# Autodesk Inventor assembly: main_assy
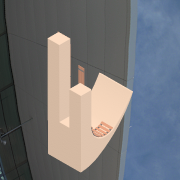
[picture p0: Inventor's stored thumbnail of the model, 180x180]
Saved by Autodesk Inventor 2019 (Build 230136000, 136)
## iProperties
Created: 2019-02-23
Part Number: main_assy
Document SubType Name: Assembly
Designer: gaincarlo
Author: gaincarlo
## Documents named in this file (9)
- D:\Giancarlo Bacchio\Documenti\00 - Progetti\30-Inventor\LaPanca-Baraca\main_assy.iam
- D:\Giancarlo Bacchio\Documenti\00 - Progetti\30-Inventor\LaPanca-Baraca\concrete_main.ipt
- D:\Giancarlo Bacchio\Documenti\00 - Progetti\30-Inventor\LaPanca-Baraca\back_plates_MIR1.iam
- D:\Giancarlo Bacchio\Documenti\00 - Progetti\30-Inventor\LaPanca-Baraca\solar_panel.ipt
- D:\Giancarlo Bacchio\Documenti\00 - Progetti\30-Inventor\LaPanca-Baraca\solar_panel_MIR.ipt
- D:\Giancarlo Bacchio\Documenti\00 - Progetti\30-Inventor\LaPanca-Baraca\curved-+_plates.iam
- D:\Giancarlo Bacchio\Documenti\00 - Progetti\30-Inventor\LaPanca-Baraca\curved-+_plates_MIR.iam
- D:\Giancarlo Bacchio\Documenti\00 - Progetti\30-Inventor\LaPanca-Baraca\support3.ipt
- D:\Giancarlo Bacchio\Documenti\00 - Progetti\30-Inventor\LaPanca-Baraca\doga_long1.ipt
## Components (13 placed, 8 different names)
1. concrete_main:1 — Flush:4
2. solar_panel:1
3. solar_panel_MIR:1
4. curved-+_plates:1 [sub-assembly] — Flush:4
5. curved-+_plates_MIR:1 [sub-assembly]
6. back_plates_MIR1:2 [sub-assembly]
7. back_plates_MIR1:3 [sub-assembly]
8. support3:1 — Mate:13, Mate:14
9. support3:2 — Mate:12
10. support3:3
11. doga_long1:1 — Mate:12, Mate:13, Mate:14
12. doga_long1:2
13. doga_long1:3
## Component patterns: (2 elements, first: back_plates_MIR1:2), (3 elements, first: support3:1), (3 elements, first: doga_long1:1)
## Relationships (4: Mate 3, Flush 1)
- Flush:4 (10 mm): concrete_main:1 ↔ curved-+_plates:1
- Mate:12: support3:2 ↔ doga_long1:1
- Mate:13: support3:1 ↔ doga_long1:1
- Mate:14: support3:1 ↔ doga_long1:1
